# Autodesk Inventor assembly: sCMOSassembly
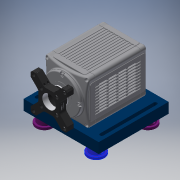
[picture p0: Inventor's stored thumbnail of the model, 180x180]
Saved by Autodesk Inventor 2016 (Build 200138000, 138)
## iProperties
Created: 2016-02-21
Part Number: sCMOSassembly
Document SubType Name: Assembly
Designer: sims01
Author: sims01
## Documents named in this file (7)
- H:\Documents\LSFM_3\setup\mechanical\design\lsfm3_mechDesign\sCMOSassembly.iam
- H:\Documents\LSFM_2\mechanicalDesign\sCMOSmountingBase.ipt
- H:\Documents\LSFM_3\setup\mechanical\design\lsfm3_mechDesign\flash4.ipt
- H:\Documents\LSFM_3\setup\mechanical\design\lsfm3_mechDesign\cMountSM1Adapter.ipt
- H:\Documents\LSFM_3\setup\mechanical\design\lsfm3_mechDesign\sm1Coupler.ipt
- H:\Documents\LSFM_3\setup\mechanical\design\lsfm3_mechDesign\30mm60mmCageAdapter.ipt
- H:\Documents\LSFM_3\setup\mechanical\design\lsfm3_mechDesign\19mmPedestalPost.ipt
## Components (9 placed, 6 different names)
1. sCMOSmountingBase:2 — Rigid:1, Rigid:9, Rigid:10, Rigid:11, Rigid:12
2. flash4:1 — Rigid:1, Rigid:6
3. cMountSM1Adapter:1 — Rigid:6, Rigid:7
4. sm1Coupler:1 — Rigid:7, Rigid:8
5. 30mm60mmCageAdapter:1 — Rigid:8
6. 19mmPedestalPost:1 — Rigid:10
7. 19mmPedestalPost:2 — Rigid:12
8. 19mmPedestalPost:3 — Rigid:11
9. 19mmPedestalPost:4 — Rigid:9
## Relationships (8: WeldJoint 8)
- Rigid:1 [WeldJoint]: sCMOSmountingBase:2 ↔ flash4:1
- Rigid:6 [WeldJoint]: flash4:1 ↔ cMountSM1Adapter:1
- Rigid:7 [WeldJoint]: cMountSM1Adapter:1 ↔ sm1Coupler:1
- Rigid:8 [WeldJoint]: sm1Coupler:1 ↔ 30mm60mmCageAdapter:1
- Rigid:9 [WeldJoint]: sCMOSmountingBase:2 ↔ 19mmPedestalPost:4
- Rigid:10 [WeldJoint]: sCMOSmountingBase:2 ↔ 19mmPedestalPost:1
- Rigid:11 [WeldJoint]: sCMOSmountingBase:2 ↔ 19mmPedestalPost:3
- Rigid:12 [WeldJoint]: sCMOSmountingBase:2 ↔ 19mmPedestalPost:2
